# Autodesk Inventor assembly: Hydraulikzylinder_mit_Befestigung_an_Platte
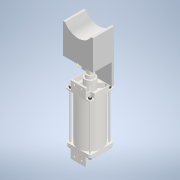
[picture p0: Inventor's stored thumbnail of the model, 180x180]
Saved by Autodesk Inventor 2020.3 (Build 243373000, 373)
## iProperties
Created: 2021-08-10
Part Number: Hydraulikzylinder_mit_Befestigung_an_Platte
Document SubType Name: Assembly
Designer: Preuß P. Ch.
Author: Preuß P. Ch.
## Documents named in this file (11)
- D:\Studium\Praegemaschine\3D-Modelle\Hydraulikzylinder_mit_Befestigung_an_Platte.iam
- C:\Users\user\Documents\Inventor\Hydraulikzylinder\Gehäuse.ipt
- C:\Users\user\Documents\Inventor\Hydraulikzylinder\Deckel_vorne_Befestigung.ipt
- C:\Users\user\Documents\Inventor\Hydraulikzylinder\Kolbenstange.ipt
- C:\Users\user\Documents\Inventor\Hydraulikzylinder\Kolben.ipt
- C:\Users\user\Documents\Inventor\Hydraulikzylinder\Gelenkflansch.ipt
- C:\Users\user\Documents\Inventor\Hydraulikzylinder\Gewindestange_360.ipt
- C:\Users\user\Documents\Inventor\Content Center Files\R2020\de-DE\ISO 4033(1)\ISO 4033 - M10DIN EN.ipt
- C:\Users\user\Documents\Inventor\Hydraulikzylinder\Ausschub_Magazin.ipt
- C:\Users\user\Documents\Inventor\Content Center Files\R2020\de-DE\ISO 4033(1)\ISO 4033 - M14DIN EN.ipt
- C:\Users\user\Documents\Inventor\Content Center Files\R2020\de-DE\DIN EN ISO 4018\DIN EN ISO 4018 - M14x50 - DIN EN ISO 4018.ipt
## Components (20 placed, 10 different names)
1. Gehäuse:1 — Passend:1, Passend:2, Passend:4, Passend:5, Passend:6, Einfügen:2, Einfügen:3, Einfügen:4, Fluchtend:1
2. Deckel_vorne_Befestigung:2 — Passend:1, Passend:2, Einfügen:1, Einfügen:5, Einfügen:6, Einfügen:7, Einfügen:8, Passend:7, Fluchtend:1, Winkel:1
3. Kolbenstange:1 — Starr:1, Passend:7, Passend:8, Einfügen:13, Winkel:1
4. Kolben:1 — Starr:1
5. Gelenkflansch:2 — Passend:4, Passend:5, Passend:6, Einfügen:9, Einfügen:10, Einfügen:11, Einfügen:12
6. Gewindestange_360:1 — Einfügen:1
7. Gewindestange_360:2 — Einfügen:2
8. Gewindestange_360:3 — Einfügen:3
9. Gewindestange_360:4 — Einfügen:4
10. DIN EN 24033 M10:3 — Einfügen:12
11. DIN EN 24033 M10:4 — Einfügen:6
12. DIN EN 24033 M10:5 — Einfügen:11
13. DIN EN 24033 M10:6 — Einfügen:5
14. DIN EN 24033 M10:7 — Einfügen:7
15. DIN EN 24033 M10:8 — Einfügen:8
16. DIN EN 24033 M10:9 — Einfügen:10
17. DIN EN 24033 M10:10 — Einfügen:9
18. Ausschub_Magazin:1 — Passend:8, Einfügen:13, Einfügen:14, Einfügen:15
19. DIN EN 24033 M14:1 — Einfügen:15
20. DIN EN ISO 4018 M14x50:1 — Einfügen:14
## Relationships (25: Insert 15, Mate 7, WeldJoint 1, Flush 1, Angle 1)
- Passend:1 [Mate]: Gehäuse:1 ↔ Deckel_vorne_Befestigung:2
- Passend:2 [Mate]: Gehäuse:1 ↔ Deckel_vorne_Befestigung:2
- Starr:1 [WeldJoint]: Kolbenstange:1 ↔ Kolben:1
- Passend:4 [Mate]: Gehäuse:1 ↔ Gelenkflansch:2
- Passend:5 [Mate]: Gehäuse:1 ↔ Gelenkflansch:2
- Passend:6 [Mate]: Gehäuse:1 ↔ Gelenkflansch:2
- Einfügen:1 [Insert] (-12.5 mm): Deckel_vorne_Befestigung:2 ↔ Gewindestange_360:1
- Einfügen:2 [Insert] (-12.5 mm): Gehäuse:1 ↔ Gewindestange_360:2
- Einfügen:3 [Insert] (-12.5 mm): Gehäuse:1 ↔ Gewindestange_360:3
- Einfügen:4 [Insert] (-12.5 mm): Gehäuse:1 ↔ Gewindestange_360:4
- Einfügen:5 [Insert]: Deckel_vorne_Befestigung:2 ↔ DIN EN 24033 M10:6
- Einfügen:6 [Insert]: Deckel_vorne_Befestigung:2 ↔ DIN EN 24033 M10:4
- Einfügen:7 [Insert]: Deckel_vorne_Befestigung:2 ↔ DIN EN 24033 M10:7
- Einfügen:8 [Insert]: Deckel_vorne_Befestigung:2 ↔ DIN EN 24033 M10:8
- Einfügen:9 [Insert]: Gelenkflansch:2 ↔ DIN EN 24033 M10:10
- Einfügen:10 [Insert]: Gelenkflansch:2 ↔ DIN EN 24033 M10:9
- Einfügen:11 [Insert]: Gelenkflansch:2 ↔ DIN EN 24033 M10:5
- Einfügen:12 [Insert]: Gelenkflansch:2 ↔ DIN EN 24033 M10:3
- Passend:7 [Mate]: Deckel_vorne_Befestigung:2 ↔ Kolbenstange:1
- Passend:8 [Mate]: Kolbenstange:1 ↔ Ausschub_Magazin:1
- Einfügen:13 [Insert]: Kolbenstange:1 ↔ Ausschub_Magazin:1
- Einfügen:14 [Insert]: Ausschub_Magazin:1 ↔ DIN EN ISO 4018 M14x50:1
- Einfügen:15 [Insert]: Ausschub_Magazin:1 ↔ DIN EN 24033 M14:1
- Fluchtend:1 [Flush]: Gehäuse:1 ↔ Deckel_vorne_Befestigung:2
- Winkel:1 [Angle] (180 deg): Deckel_vorne_Befestigung:2 ↔ Kolbenstange:1
